# Autodesk Inventor assembly: Armazon_parcial1
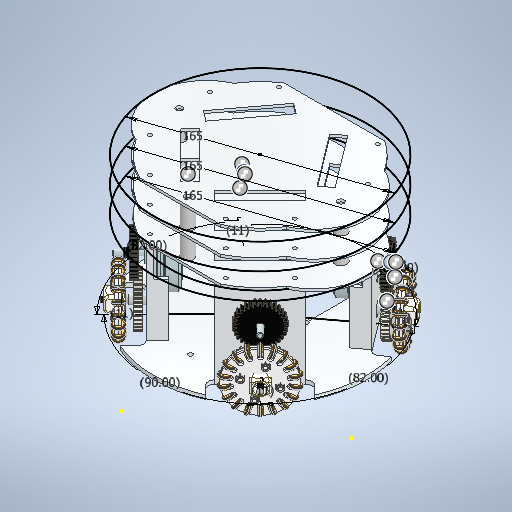
[picture p0: Inventor's stored thumbnail of the model, 512x512]
Saved by Autodesk Inventor 2025.1 (Build 291241000, 241)
## iProperties
Created: 2011-08-15
Part Number: Armazon_parcial1
Document SubType Name: Assembly
Designer: paeze
Sending System: SolidWorks 2016
Last Author: Thiago
Last Saved: 2017-11-05
Author: paeze
## Documents named in this file (10)
- J:\URUBOTS\Base_Ruedas\GITHUB\Small_Size_Robot\Armazones\Armazon_parcial1.iam
- J:\URUBOTS\Base_Ruedas\GITHUB\Small_Size_Robot\BASEmodf.ipt
- J:\URUBOTS\Base_Ruedas\GITHUB\Small_Size_Robot\Eje.ipt
- J:\URUBOTS\Base_Ruedas\GITHUB\Small_Size_Robot\Piezas de validacion\GTF Robots 50mm Wheel v4.ipt
- J:\URUBOTS\Base_Ruedas\GITHUB\Small_Size_Robot\Ruleman.ipt
- J:\URUBOTS\Base_Ruedas\GITHUB\Small_Size_Robot\Piezas de validacion\387266_ec45fl_30w_a_kabel.ipt
- J:\URUBOTS\Base_Ruedas\GITHUB\Small_Size_Robot\EngranajeChico.ipt
- J:\URUBOTS\Base_Ruedas\GITHUB\Small_Size_Robot\EngranajeGrande.ipt
- J:\URUBOTS\Base_Ruedas\GITHUB\Small_Size_Robot\Primer capa de prueba.ipt
- J:\URUBOTS\Base_Ruedas\GITHUB\Small_Size_Robot\Separador.ipt
## Components (35 placed, 9 different names)
1. BASEmodf:1 — Rigid:1, Rotational:1, Rotational:2, Rigid:4, Rotational:3, Rotational:4, Rigid:9, Rigid:10, Rotational:5, Rigid:11, Rigid:12, Rigid:21, Rigid:22
2. Eje:1 — Rigid:1, Rigid:18, Rigid:20
3. GTF Robots 50mm Wheel v4:1 — Rigid:18
4. Ruleman:1 — Rotational:1
5. Ruleman:2 — Rigid:8
6. Ruleman:3 — Rotational:4
7. Ruleman:4 — Rotational:3
8. 387266_ec45fl_30w_a_kabel:1 — Rotational:2, Rigid:5
9. Eje:2 — Rigid:4, Rigid:6, Rigid:7, Rigid:8
10. GTF Robots 50mm Wheel v4:2 — Rigid:7
11. Spur Gear1:1 — Rigid:5
12. Spur Gear2:1 — Rigid:6
13. 387266_ec45fl_30w_a_kabel:2 — Rotational:5, Rigid:16
14. 387266_ec45fl_30w_a_kabel:3 — Rigid:10, Rigid:19
15. 387266_ec45fl_30w_a_kabel:4 — Rigid:9, Rigid:13
16. Eje:3 — Rigid:11, Rigid:14, Rigid:15
17. Eje:4 — Rigid:12, Rotational:6, Rigid:17
18. Spur Gear1:4 — Rigid:13
19. Spur Gear2:2 — Rigid:14
20. GTF Robots 50mm Wheel v4:3 — Rigid:15
21. GTF Robots 50mm Wheel v4:4 — Rigid:17
22. Spur Gear1:5 — Rigid:16
23. Spur Gear2:3 — Rotational:6
24. Spur Gear1:6 — Rigid:19
25. Spur Gear2:4 — Rigid:20
26. Primer capa de prueba:1 — Rigid:21
27. Primer capa de prueba:2 — Rigid:22, Rigid:23, Rigid:24, Rigid:25
28. Separador:1 — Rigid:23, Rotational:7
29. Separador:2 — Rigid:24
30. Separador:3 — Rigid:25
31. Primer capa de prueba:3 — Rotational:7, Rigid:26, Rigid:27, Rigid:28
32. Separador:4 — Rigid:26, Rigid:29
33. Separador:5 — Rigid:27
34. Separador:6 — Rigid:28
35. Primer capa de prueba:4 — Rigid:29
## Relationships (34: WeldJoint 27, RevoluteJoint 7)
- Rigid:1 [WeldJoint] (10 mm): BASEmodf:1 ↔ Eje:1
- Rotational:1 [RevoluteJoint]: BASEmodf:1 ↔ Ruleman:1
- Rotational:2 [RevoluteJoint] (2 mm): BASEmodf:1 ↔ 387266_ec45fl_30w_a_kabel:1
- Rigid:4 [WeldJoint] (5 mm): BASEmodf:1 ↔ Eje:2
- Rigid:5 [WeldJoint]: 387266_ec45fl_30w_a_kabel:1 ↔ Spur Gear1:1
- Rigid:6 [WeldJoint] (-6 mm): Eje:2 ↔ Spur Gear2:1
- Rigid:7 [WeldJoint] (-4 mm): Eje:2 ↔ GTF Robots 50mm Wheel v4:2
- Rotational:3 [RevoluteJoint]: BASEmodf:1 ↔ Ruleman:4
- Rotational:4 [RevoluteJoint]: BASEmodf:1 ↔ Ruleman:3
- Rigid:8 [WeldJoint]: Ruleman:2 ↔ Eje:2
- Rigid:9 [WeldJoint]: BASEmodf:1 ↔ 387266_ec45fl_30w_a_kabel:4
- Rigid:10 [WeldJoint]: BASEmodf:1 ↔ 387266_ec45fl_30w_a_kabel:3
- Rotational:5 [RevoluteJoint]: BASEmodf:1 ↔ 387266_ec45fl_30w_a_kabel:2
- Rigid:11 [WeldJoint]: BASEmodf:1 ↔ Eje:3
- Rigid:12 [WeldJoint] (5 mm): BASEmodf:1 ↔ Eje:4
- Rigid:13 [WeldJoint] (5 mm): 387266_ec45fl_30w_a_kabel:4 ↔ Spur Gear1:4
- Rigid:14 [WeldJoint] (-8 mm): Eje:3 ↔ Spur Gear2:2
- Rigid:15 [WeldJoint] (-7 mm): Eje:3 ↔ GTF Robots 50mm Wheel v4:3
- Rigid:16 [WeldJoint]: 387266_ec45fl_30w_a_kabel:2 ↔ Spur Gear1:5
- Rotational:6 [RevoluteJoint]: Eje:4 ↔ Spur Gear2:3
- Rigid:17 [WeldJoint] (-2 mm): Eje:4 ↔ GTF Robots 50mm Wheel v4:4
- Rigid:18 [WeldJoint] (-8 mm): Eje:1 ↔ GTF Robots 50mm Wheel v4:1
- Rigid:19 [WeldJoint]: 387266_ec45fl_30w_a_kabel:3 ↔ Spur Gear1:6
- Rigid:20 [WeldJoint] (2 mm): Eje:1 ↔ Spur Gear2:4
- Rigid:21 [WeldJoint]: BASEmodf:1 ↔ Primer capa de prueba:1
- Rigid:22 [WeldJoint]: BASEmodf:1 ↔ Primer capa de prueba:2
- Rigid:23 [WeldJoint]: Primer capa de prueba:2 ↔ Separador:1
- Rigid:24 [WeldJoint]: Primer capa de prueba:2 ↔ Separador:2
- Rigid:25 [WeldJoint]: Primer capa de prueba:2 ↔ Separador:3
- Rotational:7 [RevoluteJoint]: Separador:1 ↔ Primer capa de prueba:3
- Rigid:26 [WeldJoint]: Primer capa de prueba:3 ↔ Separador:4
- Rigid:27 [WeldJoint]: Primer capa de prueba:3 ↔ Separador:5
- Rigid:28 [WeldJoint]: Primer capa de prueba:3 ↔ Separador:6
- Rigid:29 [WeldJoint]: Separador:4 ↔ Primer capa de prueba:4
